# Autodesk Inventor assembly: FrontWheelAssembly
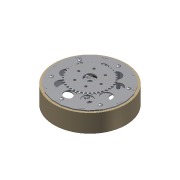
[picture p0: Inventor's stored thumbnail of the model, 180x180]
Saved by Autodesk Inventor 2012 (Build 160160000, 160)
## iProperties
Created: 2012-01-11
Part Number: FrontWheelAssembly
Document SubType Name: Assembly
Designer: JesseK
Mass: 255.836 g
Surface Area: 1707.55 cm^2
Volume: 261.441 cm^3
Density: 0.978562 g/cm^3
Author: JesseK
## Documents named in this file (4)
- Z:\UserData\Documents\Inventor\team1885frc\Robot2012\DriveTrain\FrontWheelAssembly.iam
- Z:\UserData\Documents\Inventor\team1885frc\IFI\Imported Components\IFI-WHEEL-ASSY-615-38\IFI-WHEEL-ASSY-615-38.iam
- Z:\UserData\Documents\Inventor\team1885frc\AndyMark\250-sprocket-spacer.ipt
- Z:\UserData\Documents\Inventor\team1885frc\Hardware\Sprockets\FlatSprocket_Num25_40T_0.875bore.ipt
## Components (3 placed, 3 different names)
1. IFI-WHEEL-ASSY-615-38:1 [sub-assembly] — Mate:1, Mate:2
2. 250-sprocket-spacer:1 — Mate:1, Mate:2, Mate:3, Mate:4
3. FlatSprocket_Num25_40T_0.875bore:1 — Mate:3, Mate:4
## Relationships (4: Mate 4)
- Mate:1: IFI-WHEEL-ASSY-615-38:1 ↔ 250-sprocket-spacer:1
- Mate:2: IFI-WHEEL-ASSY-615-38:1 ↔ 250-sprocket-spacer:1
- Mate:3: 250-sprocket-spacer:1 ↔ FlatSprocket_Num25_40T_0.875bore:1
- Mate:4: 250-sprocket-spacer:1 ↔ FlatSprocket_Num25_40T_0.875bore:1
